# Autodesk Inventor assembly: Antenna
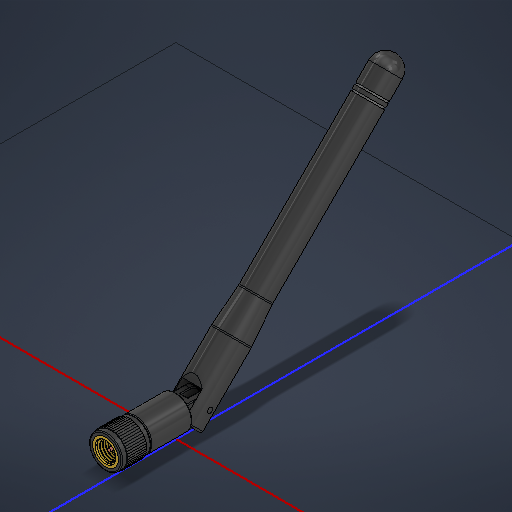
[picture p0: Inventor's stored thumbnail of the model, 512x512]
Saved by Autodesk Inventor 2025 (Build 290162000, 162)
## iProperties
Created: 2017-01-24
Part Number: Antenna
Document SubType Name: Assembly
Designer: IvanPetrov
Sending System: SolidWorks 2016
Last Author: Alexis
Last Saved: 2017-01-24
Author: IvanPetrov
## Documents named in this file (7)
- D:\Projects\OmniBot\design\standart_components\wifi antenna\Antenna\Antenna.iam
- D:\Projects\OmniBot\design\standart_components\wifi antenna\Antenna\Bottom_Radio_Antenna.ipt
- D:\Projects\OmniBot\design\standart_components\wifi antenna\Antenna\Top_Radio_Antenna.ipt
- D:\Projects\OmniBot\design\standart_components\wifi antenna\Antenna\Screw_Radio_Antenna.ipt
- D:\Projects\OmniBot\design\standart_components\wifi antenna\Antenna\Insert_Radio_Antenna.ipt
- D:\Projects\OmniBot\design\standart_components\wifi antenna\Antenna\Pin_Radio_Antenna.ipt
- D:\Projects\OmniBot\design\standart_components\wifi antenna\Antenna\Wire_Top_Radio_Antenna.ipt
## Components (7 placed, 6 different names)
1. Bottom_Radio_Antenna:2 — Совмещение:2, Угол:1
2. Top_Radio_Antenna:2 — Совмещение:1, Совмещение:2, Угол:1
3. Screw_Radio_Antenna:2
4. Insert_Radio_Antenna:2
5. Pin_Radio_Antenna:3 — Совмещение:1
6. Pin_Radio_Antenna:4
7. Wire_Top_Radio_Antenna:2
## Relationships (3: Mate 2, Angle 1)
- Совмещение:1 [Mate]: Top_Radio_Antenna:2 ↔ Pin_Radio_Antenna:3
- Совмещение:2 [Mate]: Bottom_Radio_Antenna:2 ↔ Top_Radio_Antenna:2
- Угол:1 [Angle] (-135 deg): Bottom_Radio_Antenna:2 ↔ Top_Radio_Antenna:2
